# Autodesk Inventor assembly: Assembly_XYTable_Aliepexress_cellstomr
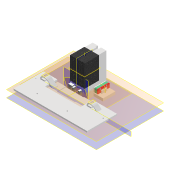
[picture p0: Inventor's stored thumbnail of the model, 180x180]
Saved by Autodesk Inventor 2022 (Build 260153000, 153)
## iProperties
Created: 2021-12-30
Part Number: Assembly_XYTable_Aliepexress_cellstomr
Document SubType Name: Assembly
Designer: diederichbenedict
Author: diederichbenedict
## Documents named in this file (7)
- C:\Users\diederichbenedict\Dropbox\Dokumente\Promotion\PROJECTS\TIRFImager\INVENTOR\Assembly_XYTable_Aliepexress_cellstomr.iam
- C:\Users\diederichbenedict\Dropbox\Dokumente\Promotion\PROJECTS\TIRFImager\INVENTOR\30_XYTabel_Aliexpress_xslide.ipt
- C:\Users\diederichbenedict\Dropbox\Dokumente\Promotion\PROJECTS\TIRFImager\INVENTOR\00_chipnano_waveguide_slidsize.ipt
- C:\Users\diederichbenedict\Dropbox\Dokumente\Promotion\PROJECTS\TIRFImager\INVENTOR\30_XYTabel_Aliexpress_cellSTORM_chiptray.ipt
- C:\Users\diederichbenedict\Dropbox\Dokumente\Promotion\PROJECTS\TIRFImager\INVENTOR\Assembly_XYTable_Aliepexress_cellstorm_laserslide.iam
- C:\Users\diederichbenedict\Dropbox\Dokumente\Promotion\PROJECTS\TIRFImager\INVENTOR\30_XYTabel_Aliexpress_cellSTORM_chiptray_spacer.ipt
- C:\Users\diederichbenedict\Dropbox\Dokumente\Promotion\PROJECTS\TIRFImager\INVENTOR\30_XYTabel_Aliexpress_cellSTORM_chiptray_clamp.ipt
## Components (7 placed, 6 different names)
1. 30_XYTabel_Aliexpress_xslide:1
2. 30_XYTabel_Aliexpress_cellSTORM_chiptray:1 — Fluchtend:11, Fluchtend:12, Einfügen:2, Einfügen:3
3. 00_chipnano_waveguide_slidsize:1
4. Assembly_XYTable_Aliepexress_cellstorm_laserslide:1 [sub-assembly]
5. 30_XYTabel_Aliexpress_cellSTORM_chiptray_spacer:1 — Fluchtend:11, Fluchtend:12
6. 30_XYTabel_Aliexpress_cellSTORM_chiptray_clamp:1 — Einfügen:2
7. 30_XYTabel_Aliexpress_cellSTORM_chiptray_clamp:2 — Einfügen:3
## Relationships (20: Flush 10, Mate 5, Insert 3, Angle 2)
- [Mate]: 30_XYTabel_Aliexpress_xslide:1 ↔ 00_chipnano_waveguide_slidsize:1
- [Mate] (15 mm): 30_XYTabel_Aliexpress_xslide:1 ↔ 00_chipnano_waveguide_slidsize:1
- [Insert] (2 mm): 00_chipnano_waveguide_slidsize:1 ↔ Assembly_XYTable_Aliepexress_cellstorm_laserslide:1
- [Angle] (0 deg): 30_XYTabel_Aliexpress_xslide:1 ↔ Assembly_XYTable_Aliepexress_cellstorm_laserslide:1
- [Mate]: 30_XYTabel_Aliexpress_xslide:1 ↔ Assembly_XYTable_Aliepexress_cellstorm_laserslide:1
- [Angle] (0 deg): 30_XYTabel_Aliexpress_xslide:1 ↔ Assembly_XYTable_Aliepexress_cellstorm_laserslide:1
- [Mate] (10 mm): 30_XYTabel_Aliexpress_xslide:1 ↔ Assembly_XYTable_Aliepexress_cellstorm_laserslide:1
- [Mate] (1 mm): 30_XYTabel_Aliexpress_xslide:1 ↔ Assembly_XYTable_Aliepexress_cellstorm_laserslide:1
- [Flush] (4 mm): 30_XYTabel_Aliexpress_xslide:1 ↔ Assembly_XYTable_Aliepexress_cellstorm_laserslide:1
- [Flush]: 30_XYTabel_Aliexpress_xslide:1 ↔ Assembly_XYTable_Aliepexress_cellstorm_laserslide:1
- [Flush]: 30_XYTabel_Aliexpress_xslide:1 ↔ Assembly_XYTable_Aliepexress_cellstorm_laserslide:1
- [Flush]: 30_XYTabel_Aliexpress_xslide:1 ↔ 30_XYTabel_Aliexpress_cellSTORM_chiptray:1
- [Flush]: 30_XYTabel_Aliexpress_xslide:1 ↔ 30_XYTabel_Aliexpress_cellSTORM_chiptray:1
- [Flush]: 30_XYTabel_Aliexpress_xslide:1 ↔ Assembly_XYTable_Aliepexress_cellstorm_laserslide:1
- [Flush]: 30_XYTabel_Aliexpress_xslide:1 ↔ Assembly_XYTable_Aliepexress_cellstorm_laserslide:1
- [Flush]: 30_XYTabel_Aliexpress_xslide:1 ↔ Assembly_XYTable_Aliepexress_cellstorm_laserslide:1
- Fluchtend:11 [Flush]: 30_XYTabel_Aliexpress_cellSTORM_chiptray:1 ↔ 30_XYTabel_Aliexpress_cellSTORM_chiptray_spacer:1
- Fluchtend:12 [Flush]: 30_XYTabel_Aliexpress_cellSTORM_chiptray:1 ↔ 30_XYTabel_Aliexpress_cellSTORM_chiptray_spacer:1
- Einfügen:2 [Insert]: 30_XYTabel_Aliexpress_cellSTORM_chiptray:1 ↔ 30_XYTabel_Aliexpress_cellSTORM_chiptray_clamp:1
- Einfügen:3 [Insert]: 30_XYTabel_Aliexpress_cellSTORM_chiptray:1 ↔ 30_XYTabel_Aliexpress_cellSTORM_chiptray_clamp:2
